# Autodesk Inventor assembly: 1. Prototype Plate Assembly
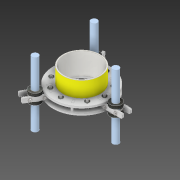
[picture p0: Inventor's stored thumbnail of the model, 180x180]
Saved by Autodesk Inventor 2020.1 (Build 241239000, 239)
## iProperties
Created: 2019-08-27
Part Number: 1. Prototype Plate Assembly
Document SubType Name: Assembly
Designer: Oliver Frolovs
Mass: 8908.37 g
Surface Area: 4981.48 cm^2
Volume: 1825.2 cm^3
Density: 4.88078 g/cm^3
Author: Oliver Frolovs
## Documents named in this file (12)
- C:\Local\prototype-plate\1. Prototype Plate Assembly.iam
- C:\Local\prototype-plate\Prototype Plate Base.ipt
- C:\Local\prototype-plate\Inner Rib.ipt
- C:\Local\prototype-plate\0. All Parameters.ipt
- C:\Local\prototype-plate\Outer Rib.ipt
- C:\Local\prototype-plate\Locate Rig Columns.ipt
- C:\Local\prototype-plate\Stator Metal Ring.ipt
- C:\Local\prototype-plate\Prototype Plate Base_MIR.ipt
- C:\Local\prototype-plate\Two Piece Clamp Huco Stock No 046201030 Dim 30-54-15.ipt
- C:\Local\prototype-plate\1. Prototype Plate Assembly\Design Accelerator\Bolted Connection Between Plate Bases.iam
- C:\Local\prototype-plate\1. Prototype Plate Assembly\Design Accelerator\Bolted Connection Plates to Arms.iam
- C:\Local\prototype-plate\1. Prototype Plate Assembly\Design Accelerator\Bolted Connection Arms Parallel Plates Together.iam
## Components (24 placed, 10 different names)
1. Prototype Plate Base:1 — Rigid:3, Rigid:5, Rigid:6, Rigid:8, Rigid:9, Mate:13, Mate:15
2. Locate Rig Columns:1 — Flush:1, Cylindrical:1
3. Stator Metal Ring:1 — Rigid:8
4. Prototype Plate Base_MIR:1 — Rigid:9, Mate:12, Mate:14
5. Bolt Plates Together [sub-assembly] — Mate:12, Mate:13
6. Bolt Arms to Plate [sub-assembly] — Mate:14, Mate:15
7. Inner Rib — Rigid:3
8. Inner Rib:2
9. Inner Rib:3
10. Outer Rib:1 — Rigid:5
11. Outer Rib:2 — Rigid:6, Mate:1, Mate:16, Mate:17
12. Outer Rib:3
13. Outer Rib:4
14. Outer Rib:5
15. Outer Rib:6
16. Bolted Connection:3 [sub-assembly] — Mate:16, Mate:17
17. Bolted Connection:4 [sub-assembly]
18. Bolted Connection:5 [sub-assembly]
19. Two Piece Clamp Huco Stock No 046201030 Dim 30-54-15:1 — Cylindrical:1, Mate:1
20. Two Piece Clamp Huco Stock No 046201030 Dim 30-54-15:2
21. Two Piece Clamp Huco Stock No 046201030 Dim 30-54-15:3
22. Two Piece Clamp Huco Stock No 046201030 Dim 30-54-15:4
23. Two Piece Clamp Huco Stock No 046201030 Dim 30-54-15:5
24. Two Piece Clamp Huco Stock No 046201030 Dim 30-54-15:6
## Component patterns: Inner Ribs (3 elements), Outer Ribs (3 elements), Two Piece Clamps to Hold the Stator (3 elements), Bolt Arms to Columns (3 elements), (2 elements, first: Two Piece Clamp Huco Stock No 046201030 Dim 30-54-15:1), Component Pattern 4:2 (2 elements), Component Pattern 4:3 (2 elements)
## Relationships (14: Mate 7, WeldJoint 5, Flush 1, CylindricalJoint 1)
- Rigid:3 [WeldJoint]: Prototype Plate Base:1 ↔ Inner Rib
- Rigid:5 [WeldJoint]: Prototype Plate Base:1 ↔ Outer Rib:1
- Rigid:6 [WeldJoint]: Prototype Plate Base:1 ↔ Outer Rib:2
- Flush:1: Locate Rig Columns:1
- Rigid:8 [WeldJoint]: Prototype Plate Base:1 ↔ Stator Metal Ring:1
- Rigid:9 [WeldJoint] (20 mm): Prototype Plate Base:1 ↔ Prototype Plate Base_MIR:1
- Cylindrical:1: Locate Rig Columns:1 ↔ Two Piece Clamp Huco Stock No 046201030 Dim 30-54-15:1
- Mate:1: Outer Rib:2 ↔ Two Piece Clamp Huco Stock No 046201030 Dim 30-54-15:1
- Mate:12: Prototype Plate Base_MIR:1 ↔ Bolt Plates Together
- Mate:13: Prototype Plate Base:1 ↔ Bolt Plates Together
- Mate:14: Prototype Plate Base_MIR:1 ↔ Bolt Arms to Plate
- Mate:15: Prototype Plate Base:1 ↔ Bolt Arms to Plate
- Mate:16: Outer Rib:2 ↔ Bolted Connection:3
- Mate:17: Outer Rib:2 ↔ Bolted Connection:3
## Named parameters: InnerRibHeight = 20 mm, RigColumnsPCD = 328 mm, RigColumnsDiameter = 30 mm, PrototypeStatorMetalRingOuterDiameter = 179.5 mm, PrototypeStatorMetalRingThickness = 5.75 mm, PrototypeStatorMetalRingHeight = 104.1 mm, TwoPieceClampOuterDiameter = 54 mm, LaserCutterKerf_MDF_9mm = 0.2 mm
